(part 1 of 2)
# Autodesk Inventor assembly: gasienica_zlozenie
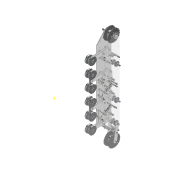
[picture p0: Inventor's stored thumbnail of the model, 180x180]
Saved by Autodesk Inventor 2020.3 (Build 243373000, 373)
## iProperties
Created: 2021-10-24
Part Number: gasienica_zlozenie
Document SubType Name: Assembly
Designer: Patryk Szydlik
Project: Projekt gąsienicowego układu jezdnego robota mobilnego "Ariadna"
Description: Projekt gąsienicowego układu jezdnego robota mobilnego "Ariadna"
Author: Patryk Szydlik
Title: Projekt gąsienicowego układu jezdnego robota mobilnego "Ariadna"
Subject: Projekt gąsienicowego układu jezdnego robota mobilnego "Ariadna"
## Documents named in this file (46)
- C:\Users\patry\Desktop\Semestr 7\Inzynierka\Projekt inventor\Ariadna_inzynierka\Workspaces\Obszar roboczy\Obszar roboczy\Naped\Zawieszenie_v3\gasienica_zlozenie.iam
- C:\Users\patry\Desktop\Semestr 7\Inzynierka\Projekt inventor\Ariadna_inzynierka\Workspaces\Obszar roboczy\Obszar roboczy\Naped\Kola\kolo_przednie.iam
- C:\Users\patry\Desktop\Semestr 7\Inzynierka\Projekt inventor\Ariadna_inzynierka\Workspaces\Obszar roboczy\Obszar roboczy\Naped\Sruby\M5_nut_5mm.ipt
- C:\Users\patry\Desktop\Semestr 7\Inzynierka\Projekt inventor\Ariadna_inzynierka\Workspaces\Obszar roboczy\Obszar roboczy\Naped\Zawieszenie_v3\tuleja_TUF106040.ipt
- C:\Users\patry\Desktop\Semestr 7\Inzynierka\Projekt inventor\Ariadna_inzynierka\Workspaces\Obszar roboczy\Obszar roboczy\Naped\Sruby\M6_nut_5mm.ipt
- C:\Users\patry\Desktop\Semestr 7\Inzynierka\Projekt inventor\Ariadna_inzynierka\Workspaces\Obszar roboczy\Obszar roboczy\Naped\Amortyzator\Korpus.ipt
- C:\Users\patry\Desktop\Semestr 7\Inzynierka\Projekt inventor\Ariadna_inzynierka\Workspaces\Obszar roboczy\Obszar roboczy\Naped\Amortyzator\Tlok.ipt
- C:\Users\patry\Desktop\Semestr 7\Inzynierka\Projekt inventor\Ariadna_inzynierka\Workspaces\Obszar roboczy\Obszar roboczy\Naped\Amortyzator\Nakretka.ipt
- C:\Users\patry\Desktop\Semestr 7\Inzynierka\Projekt inventor\Ariadna_inzynierka\Workspaces\Obszar roboczy\Obszar roboczy\Naped\Sruby\M8_nut_6.5mm_MIR1.ipt
- C:\Users\patry\Desktop\Semestr 7\Inzynierka\Projekt inventor\Ariadna_inzynierka\Workspaces\Obszar roboczy\Obszar roboczy\Naped\Sruby\M8x80_threaded_MIR1.ipt
- C:\Users\patry\Desktop\Semestr 7\Inzynierka\Projekt inventor\Ariadna_inzynierka\Workspaces\Obszar roboczy\Obszar roboczy\Naped\Sruby\M8_pad_MIR1.ipt
- C:\Users\patry\Desktop\Semestr 7\Inzynierka\Projekt inventor\Ariadna_inzynierka\Workspaces\Obszar roboczy\Obszar roboczy\Naped\Lozyska\608ZZ-8mm\bearings-608zz-80018-1.snapshot.1\608zz_MIR1.ipt
- C:\Users\patry\Desktop\Semestr 7\Inzynierka\Projekt inventor\Ariadna_inzynierka\Workspaces\Obszar roboczy\Obszar roboczy\Naped\Kola\kolo_napedowe.iam
- C:\Users\patry\Desktop\Semestr 7\Inzynierka\Projekt inventor\Ariadna_inzynierka\Workspaces\Obszar roboczy\Obszar roboczy\Naped\Sruby\M5_70_shaft.ipt
- C:\Users\patry\Desktop\Semestr 7\Inzynierka\Projekt inventor\Ariadna_inzynierka\Workspaces\Obszar roboczy\Obszar roboczy\Naped\Sruby\M3_16_shaft.ipt
- C:\Users\patry\Desktop\Semestr 7\Inzynierka\Projekt inventor\Ariadna_inzynierka\Workspaces\Obszar roboczy\Obszar roboczy\Naped\Sruby\M3_nut_2,5mm.ipt
- C:\Users\patry\Desktop\Semestr 7\Inzynierka\Projekt inventor\Ariadna_inzynierka\Workspaces\Obszar roboczy\Obszar roboczy\Naped\Zawieszenie_v3\wspornik_amortyzatora.ipt
- C:\Users\patry\Desktop\Semestr 7\Inzynierka\Projekt inventor\Ariadna_inzynierka\Workspaces\Obszar roboczy\Obszar roboczy\Naped\Sruby\M6_70_shaft.ipt
- C:\Users\patry\Desktop\Semestr 7\Inzynierka\Projekt inventor\Ariadna_inzynierka\Workspaces\Obszar roboczy\Obszar roboczy\Naped\Sruby\tuleja_M5_M9_20.ipt
- C:\Users\patry\Desktop\Semestr 7\Inzynierka\Projekt inventor\Ariadna_inzynierka\Workspaces\Obszar roboczy\Obszar roboczy\Naped\Sruby\tuleja_M5_M9_25.ipt
- C:\Users\patry\Desktop\Semestr 7\Inzynierka\Projekt inventor\Ariadna_inzynierka\Workspaces\Obszar roboczy\Obszar roboczy\Naped\Kola\holder_wheel_pair.iam
- C:\Users\patry\Desktop\Semestr 7\Inzynierka\Projekt inventor\Ariadna_inzynierka\Workspaces\Obszar roboczy\Obszar roboczy\Naped\Zawieszenie_v3\ramie_napinacza.ipt
- C:\Users\patry\Desktop\Semestr 7\Inzynierka\Projekt inventor\Ariadna_inzynierka\Workspaces\Obszar roboczy\Obszar roboczy\Naped\Sruby\M5_60_shaft.ipt
- C:\Users\patry\Desktop\Semestr 7\Inzynierka\Projekt inventor\Ariadna_inzynierka\Workspaces\Obszar roboczy\Obszar roboczy\Naped\Sruby\tuleja_M5_M9_13.ipt
- C:\Users\patry\Desktop\Semestr 7\Inzynierka\Projekt inventor\Ariadna_inzynierka\Workspaces\Obszar roboczy\Obszar roboczy\Naped\Sruby\tuleja_M5_M9_18.ipt
- C:\Users\patry\Desktop\Semestr 7\Inzynierka\Projekt inventor\Ariadna_inzynierka\Workspaces\Obszar roboczy\Obszar roboczy\Naped\Sruby\tuleja_M6_M10_8.ipt
- C:\Users\patry\Desktop\Semestr 7\Inzynierka\Projekt inventor\Ariadna_inzynierka\Workspaces\Obszar roboczy\Obszar roboczy\Naped\Zawieszenie_v3\plyta_boczna.ipt
- C:\Users\patry\Desktop\Semestr 7\Inzynierka\Projekt inventor\Ariadna_inzynierka\Workspaces\Obszar roboczy\Obszar roboczy\Naped\Zawieszenie_v3\ramie_1_wahacza.ipt
- C:\Users\patry\Desktop\Semestr 7\Inzynierka\Projekt inventor\Ariadna_inzynierka\Workspaces\Obszar roboczy\Obszar roboczy\Naped\Zawieszenie_v3\ramie_2_wahacza.ipt
- C:\Users\patry\Desktop\Semestr 7\Inzynierka\Projekt inventor\Ariadna_inzynierka\Workspaces\Obszar roboczy\Obszar roboczy\Naped\Sruby\M6_40_shaft.ipt
- C:\Users\patry\Desktop\Semestr 7\Inzynierka\Projekt inventor\Ariadna_inzynierka\Workspaces\Obszar roboczy\Obszar roboczy\Naped\Sruby\tuleja_M6_M10_7.ipt
- C:\Users\patry\Desktop\Semestr 7\Inzynierka\Projekt inventor\Ariadna_inzynierka\Workspaces\Obszar roboczy\Obszar roboczy\Naped\Sruby\M6_1,25_pad.ipt
- C:\Users\patry\Desktop\Semestr 7\Inzynierka\Projekt inventor\Ariadna_inzynierka\Workspaces\Obszar roboczy\Obszar roboczy\Naped\Sruby\M5_40_shaft.ipt
- M5_shaft.ipt
- C:\Users\patry\Desktop\Semestr 7\Inzynierka\Projekt inventor\Ariadna_inzynierka\Workspaces\Obszar roboczy\Obszar roboczy\Naped\Sruby\tuleja_M5_M9_4,5.ipt
- C:\Users\patry\Desktop\Semestr 7\Inzynierka\Projekt inventor\Ariadna_inzynierka\Workspaces\Obszar roboczy\Obszar roboczy\Naped\Zawieszenie_v3\glowny_wahacz_zewn.ipt
- C:\Users\patry\Desktop\Semestr 7\Inzynierka\Projekt inventor\Ariadna_inzynierka\Workspaces\Obszar roboczy\Obszar roboczy\Naped\Zawieszenie_v3\independent_wheel_pair.iam
- C:\Users\patry\Desktop\Semestr 7\Inzynierka\Projekt inventor\Ariadna_inzynierka\Workspaces\Obszar roboczy\Obszar roboczy\Naped\Sruby\tuleja_M6_M10_6.ipt
- C:\Users\patry\Desktop\Semestr 7\Inzynierka\Projekt inventor\Ariadna_inzynierka\Workspaces\Obszar roboczy\Obszar roboczy\Naped\Sruby\tuleja_M5_M9_17.5.ipt
- C:\Users\patry\Desktop\Semestr 7\Inzynierka\Projekt inventor\Ariadna_inzynierka\Workspaces\Obszar roboczy\Obszar roboczy\Naped\Zawieszenie_v3\komplet_kol_V4.iam
- C:\Users\patry\Desktop\Semestr 7\Inzynierka\Projekt inventor\Ariadna_inzynierka\Workspaces\Obszar roboczy\Obszar roboczy\Naped\Sruby\M6_25_shaft.ipt
- C:\Users\patry\Desktop\Semestr 7\Inzynierka\Projekt inventor\Ariadna_inzynierka\Workspaces\Obszar roboczy\Obszar roboczy\Naped\Kola\single_wheel_dummie.iam
- C:\Users\patry\Desktop\Semestr 7\Inzynierka\Projekt inventor\Ariadna_inzynierka\Workspaces\Obszar roboczy\Obszar roboczy\Naped\Sruby\tuleja_M5_M10_15.ipt
- C:\Users\patry\Desktop\Semestr 7\Inzynierka\Projekt inventor\Ariadna_inzynierka\Workspaces\Obszar roboczy\Obszar roboczy\Naped\Sruby\tuleja_M6_M10_7,5.ipt
- C:\Users\patry\Desktop\Semestr 7\Inzynierka\Projekt inventor\Ariadna_inzynierka\Workspaces\Obszar roboczy\Obszar roboczy\Naped\Zawieszenie_v3\ramie_2_wahacza_tylnego.ipt
- C:\Users\patry\Desktop\Semestr 7\Inzynierka\Projekt inventor\Ariadna_inzynierka\Workspaces\Obszar roboczy\Obszar roboczy\Naped\Sruby\M6x25_plaski_leb.ipt
## Components (343 placed, 44 different names)
1. M8_nut_6.5mm_MIR1:1
2. M8x80_threaded_MIR1:1
3. M8_nut_6.5mm_MIR1:2
4. M8_nut_6.5mm_MIR1:3
5. M8_pad_MIR1:1
6. M8_pad_MIR1:2
7. M8_pad_MIR1:3
8. M8_pad_MIR1:4
9. 608zz_MIR1:1
10. 608zz_MIR1:2 — Zestawiające:1077, Równoległe:74
11. kolo_napedowe:1 [sub-assembly]
12. kolo_przednie:1 [sub-assembly]
13. ramie_napinacza:1 — Zestawiające:1807
14. Korpus:6 — Walcowe:6
15. Tlok:6 — Walcowe:6
16. Nakretka:6
17. M5_nut_5mm:34
18. M5_70_shaft:6 — Zestawiające:1080
19. M5_nut_5mm:35
20. M3_16_shaft:6
21. M3_nut_2,5mm:11
22. M3_nut_2,5mm:12
23. wspornik_amortyzatora:11 — Zestawiające:1086, Zestawiające:1087
24. wspornik_amortyzatora:12
25. M5_nut_5mm:36
26. M5_nut_5mm:37
27. M5_nut_5mm:38
28. M5_nut_5mm:39
29. tuleja_M5_M9_20:6
30. tuleja_M5_M9_25:6
31. ramie_napinacza:2 — Zestawiające:1804
32. M5_60_shaft:1 — Zestawiające:1086
33. M5_60_shaft:2 — Zestawiające:1087, Zestawiające:1796, Zestawiające:1797
34. tuleja_TUF106040:41 — Zestawiające:1085
35. tuleja_TUF106040:42
36. M6_70_shaft:11 — Zestawiające:1079, Zestawiające:1802, Zestawiające:1803, Zestawiające:1806
37. M6_nut_5mm:49
38. M6_nut_5mm:50
39. tuleja_M5_M9_13:1 — Zestawiające:1796
40. tuleja_M5_M9_18:1 — Zestawiające:1797
41. M6_70_shaft:12
42. M6_nut_5mm:51
43. M6_nut_5mm:52
44. tuleja_M6_M10_8:1
45. tuleja_M6_M10_8:2
46. holder_wheel_pair:4 [sub-assembly] — Zestawiające:1082, Zestawiające:1083
47. holder_wheel_pair:5 [sub-assembly] — Zestawiające:1081, Zestawiające:1084
48. plyta_boczna:1 — Zestawiające:1075, Zestawiające:1076, Zestawiające:1077, Zestawiające:1078, Równoległe:74, Kątowe:22, Zestawiające:1079, Zestawiające:1080, Zestawiające:1081, Zestawiające:1082, Zestawiające:1083, Zestawiające:1084, Zestawiające:1085, Zestawiające:1632, Zestawiające:1633, Kątowe:49, Zestawiające:1950, Zestawiające:1951, Zestawiające:1952, Zestawiające:1953
49. plyta_boczna:2 — Zestawiające:1075, Zestawiające:1076, Zestawiające:1078, Zestawiające:1636, Zestawiające:1637, Zestawiające:1638, Zestawiające:1639, Zestawiające:1640, Zestawiające:1641, Zestawiające:1777, Zestawiające:1778, Zestawiające:1779, Zestawiające:1780
50. ramie_1_wahacza:3
51. ramie_2_wahacza:3
52. tuleja_TUF106040:51
53. tuleja_TUF106040:52
54. tuleja_TUF106040:53
55. tuleja_TUF106040:54
56. tuleja_TUF106040:55
57. tuleja_TUF106040:56
58. ramie_2_wahacza:4
59. tuleja_TUF106040:57
60. tuleja_TUF106040:58
61. M6_nut_5mm:65
62. Korpus:8
63. Tlok:8
64. Nakretka:8
65. M5_nut_5mm:48
66. M5_70_shaft:8
67. ramie_1_wahacza:4 — Kątowe:40
68. M5_nut_5mm:49
69. M3_16_shaft:8
70. M3_nut_2,5mm:15
71. M3_nut_2,5mm:16
72. wspornik_amortyzatora:15
73. wspornik_amortyzatora:16
74. M6_40_shaft:3
75. M6_40_shaft:4
76. M6_nut_5mm:66
77. M6_nut_5mm:67
78. M6_nut_5mm:68
79. tuleja_M6_M10_7:4
80. tuleja_M6_M10_7:5
81. M6_1,25_pad:9
82. M6_1,25_pad:10
83. M6_1,25_pad:11
84. M6_1,25_pad:12
85. M6_1,25_pad:13
86. M6_1,25_pad:14
87. M6_1,25_pad:15
88. M6_1,25_pad:16
89. M6_70_shaft:15 — Zestawiające:1636
90. M6_70_shaft:16 — Zestawiające:1632
91. M6_nut_5mm:69
92. M6_nut_5mm:70
93. M6_nut_5mm:71
94. M6_nut_5mm:72
95. M5_shaft:3
96. M5_shaft:4
97. M5_nut_5mm:50
98. M5_nut_5mm:51
99. M5_nut_5mm:52
100. M5_nut_5mm:53
101. tuleja_M5_M9_4,5:5
102. tuleja_M5_M9_4,5:6
103. tuleja_M5_M9_4,5:7
104. tuleja_M5_M9_4,5:8
105. lacznik_zewn:3 — Kątowe:40, Zestawiające:1793, Zestawiające:1794, Zestawiające:1795
106. lacznik_zewn:4 — Zestawiające:1793
107. tuleja_M6_M10_6:5
108. M6_nut_5mm:73
109. M6_nut_5mm:74
110. M6_nut_5mm:75 — Zestawiające:1633
111. M6_nut_5mm:76
112. tuleja_M6_M10_6:6
113. tuleja_M6_M10_6:7
114. tuleja_M6_M10_6:8
115. M5_nut_5mm:54
116. M5_nut_5mm:55
117. tuleja_M5_M9_17.5:3 — Zestawiające:1637
118. tuleja_M5_M9_17.5:4
119. ramie_1_wahacza:7 — Kątowe:41
120. ramie_2_wahacza:7
121. tuleja_TUF106040:67
122. tuleja_TUF106040:68
123. tuleja_TUF106040:69
124. tuleja_TUF106040:70
125. tuleja_TUF106040:71
126. tuleja_TUF106040:72
127. ramie_2_wahacza:8
128. tuleja_TUF106040:73
129. tuleja_TUF106040:74
130. M6_nut_5mm:89
131. Korpus:10 — Walcowe:10
132. Tlok:10 — Walcowe:10
133. Nakretka:10
134. M5_nut_5mm:64
135. M5_70_shaft:10
136. ramie_1_wahacza:8
137. M5_nut_5mm:65 — Zestawiające:1638
138. M3_16_shaft:10
139. M3_nut_2,5mm:19
140. M3_nut_2,5mm:20
141. wspornik_amortyzatora:19
142. wspornik_amortyzatora:20
143. M6_40_shaft:7
144. M6_40_shaft:8
145. M6_nut_5mm:90
146. M6_nut_5mm:91
147. M6_nut_5mm:92
148. tuleja_M6_M10_7:10
149. tuleja_M6_M10_7:11
150. M6_1,25_pad:25
151. M6_1,25_pad:26
152. M6_1,25_pad:27
153. M6_1,25_pad:28
154. M6_1,25_pad:29
155. M6_1,25_pad:30
156. M6_1,25_pad:31
157. M6_1,25_pad:32
158. M6_70_shaft:19 — Zestawiające:1640
159. M6_70_shaft:20 — Zestawiające:1639
160. M6_nut_5mm:93
161. M6_nut_5mm:94
162. M6_nut_5mm:95
163. M6_nut_5mm:96
164. M5_shaft:7
165. M5_shaft:8
166. M5_nut_5mm:66
167. M5_nut_5mm:67
168. M5_nut_5mm:68
169. M5_nut_5mm:69
170. tuleja_M5_M9_4,5:13
171. tuleja_M5_M9_4,5:14
172. tuleja_M5_M9_4,5:15
173. tuleja_M5_M9_4,5:16
174. lacznik_zewn:7 — Zestawiające:1784
175. lacznik_zewn:8 — Kątowe:41, Zestawiające:1781, Zestawiające:1782, Zestawiające:1789
176. tuleja_M6_M10_6:13
177. M6_nut_5mm:97
178. M6_nut_5mm:98
179. M6_nut_5mm:99
180. M6_nut_5mm:100
181. tuleja_M6_M10_6:14
182. tuleja_M6_M10_6:15
183. tuleja_M6_M10_6:16
184. M5_nut_5mm:70
185. M5_nut_5mm:71
186. tuleja_M5_M9_17.5:7 — Zestawiające:1641
187. tuleja_M5_M9_17.5:8
188. ramie_1_wahacza:9 — Kątowe:47
189. ramie_2_wahacza:9
190. tuleja_TUF106040:75
191. tuleja_TUF106040:76
192. tuleja_TUF106040:77
193. tuleja_TUF106040:78
194. tuleja_TUF106040:79
195. tuleja_TUF106040:80
196. ramie_2_wahacza:10
197. tuleja_TUF106040:81
198. tuleja_TUF106040:82
199. M6_nut_5mm:101
200. Korpus:11 — Walcowe:11
201. Tlok:11 — Walcowe:11
202. Nakretka:11
203. M5_nut_5mm:72
204. M5_70_shaft:11
205. ramie_1_wahacza:10
206. M5_nut_5mm:73
207. M3_16_shaft:11
208. M3_nut_2,5mm:21
209. M3_nut_2,5mm:22
210. wspornik_amortyzatora:21
211. wspornik_amortyzatora:22
212. M6_40_shaft:9
213. M6_40_shaft:10
214. M6_nut_5mm:102
215. M6_nut_5mm:103
216. M6_nut_5mm:104
217. tuleja_M6_M10_7:13
218. tuleja_M6_M10_7:14
219. M6_1,25_pad:33
220. M6_1,25_pad:34
221. M6_1,25_pad:35
222. M6_1,25_pad:36
223. M6_1,25_pad:37
224. M6_1,25_pad:38
225. M6_1,25_pad:39
226. M6_1,25_pad:40
227. M6_70_shaft:21 — Zestawiające:1779
228. M6_70_shaft:22 — Zestawiające:1778
229. M6_nut_5mm:105
230. M6_nut_5mm:106
231. M6_nut_5mm:107 — Zestawiające:1777
232. M6_nut_5mm:108
233. M5_shaft:9
234. M5_shaft:10
235. M5_nut_5mm:74
236. M5_nut_5mm:75
237. M5_nut_5mm:76
238. M5_nut_5mm:77
239. tuleja_M5_M9_4,5:17
240. tuleja_M5_M9_4,5:18
241. tuleja_M5_M9_4,5:19
242. tuleja_M5_M9_4,5:20
243. lacznik_zewn:9
244. lacznik_zewn:10 — Kątowe:47
245. independent_wheel_pair:5 [sub-assembly]
246. tuleja_M6_M10_7:15
247. tuleja_M6_M10_6:17
248. M6_nut_5mm:109
249. M6_nut_5mm:110
250. M6_nut_5mm:111
251. M6_nut_5mm:112
252. tuleja_M6_M10_6:18
253. tuleja_M6_M10_6:19
254. tuleja_M6_M10_6:20
255. M5_nut_5mm:78
256. M5_nut_5mm:79
257. tuleja_M5_M9_17.5:9
258. tuleja_M5_M9_17.5:10 — Zestawiające:1780
259. komplet_kol_V4:1 [sub-assembly] — Zestawiające:1781, Zestawiające:1782, Zestawiające:1784, Zestawiające:1788, Kątowe:48
260. M6_nut_5mm:115 — Zestawiające:1789
261. M6_25_shaft:2 — Zestawiające:1788
262. M6_nut_5mm:116
263. komplet_kol_V4:2 [sub-assembly] — Zestawiające:1795, Kątowe:48, Kątowe:49, Styczny:1
264. M6_nut_5mm:117
265. M6_25_shaft:3 — Zestawiające:1794
266. M6_nut_5mm:118
267. single_wheel_dummie:1 [sub-assembly] — Zestawiające:1799
268. single_wheel_dummie:2 [sub-assembly] — Zestawiające:1800, Zestawiające:1801, Zestawiające:1802, Zestawiające:1805
269. tuleja_M5_M10_15:1 — Zestawiające:1799, Zestawiające:1800, Zestawiające:1801
270. tuleja_M6_M10_7,5:1 — Zestawiające:1803, Zestawiające:1804, Zestawiające:1805
271. tuleja_M6_M10_7,5:2 — Zestawiające:1806, Zestawiające:1807
272. ramie_1_wahacza:11
273. tuleja_TUF106040:83
274. tuleja_TUF106040:84
275. tuleja_TUF106040:85
276. tuleja_TUF106040:86
277. tuleja_TUF106040:87
278. tuleja_TUF106040:88
279. tuleja_TUF106040:89
280. tuleja_TUF106040:90
281. M6_nut_5mm:119
282. Korpus:12 — Walcowe:12
283. Tlok:12 — Walcowe:12
284. Nakretka:12
285. M5_nut_5mm:80
286. M5_70_shaft:12
287. ramie_1_wahacza:12
288. M5_nut_5mm:81
289. M3_16_shaft:12
290. M3_nut_2,5mm:23
291. M3_nut_2,5mm:24
292. wspornik_amortyzatora:23
293. wspornik_amortyzatora:24
294. M6_40_shaft:11
295. M6_40_shaft:12
296. M6_nut_5mm:120
297. M6_nut_5mm:121
298. M6_nut_5mm:122
299. tuleja_M6_M10_7:16
300. tuleja_M6_M10_7:17
301. M6_1,25_pad:41
302. M6_1,25_pad:42
303. M6_1,25_pad:43
304. M6_1,25_pad:44
305. M6_1,25_pad:45
306. M6_1,25_pad:46
307. M6_1,25_pad:47
308. M6_1,25_pad:48
309. M6_70_shaft:23 — Zestawiające:1950
310. M6_nut_5mm:123 — Zestawiające:1951
311. M6_nut_5mm:124
312. M6_nut_5mm:125
313. M6_nut_5mm:126
314. M5_shaft:11
315. M5_shaft:12
316. M5_nut_5mm:82
317. M5_nut_5mm:83
318. M5_nut_5mm:84
319. M5_nut_5mm:85
320. tuleja_M5_M9_4,5:21
321. tuleja_M5_M9_4,5:22
322. tuleja_M5_M9_4,5:23
323. tuleja_M5_M9_4,5:24
324. lacznik_zewn:11
325. lacznik_zewn:12
326. independent_wheel_pair:6 [sub-assembly] — Styczny:1
327. tuleja_M6_M10_7:18
328. tuleja_M6_M10_6:21
329. M6_nut_5mm:127
330. M6_nut_5mm:128
331. M6_nut_5mm:129
332. M6_nut_5mm:130
333. tuleja_M6_M10_6:22 — Zestawiające:1952
334. tuleja_M6_M10_6:23
335. tuleja_M6_M10_6:24
336. M5_nut_5mm:86
337. M5_nut_5mm:87
338. tuleja_M5_M9_17.5:11
339. tuleja_M5_M9_17.5:12 — Zestawiające:1953
340. ramie_2_wahacza_tylnego:1
341. ramie_2_wahacza_tylnego:2
342. M6x25_plaski_leb:1
343. M6x25_plaski_leb:2
## Relationships (738: Mate 664, Flush 48, Angle 21, CylindricalJoint 4, Tangent 1)
- [Mate]: M8_nut_6.5mm_MIR1:1 ↔ M8x80_threaded_MIR1:1
- [Mate]: M8x80_threaded_MIR1:1 ↔ M8_nut_6.5mm_MIR1:2
- [Mate]: M8x80_threaded_MIR1:1 ↔ M8_nut_6.5mm_MIR1:3
- [Mate]: M8_nut_6.5mm_MIR1:1 ↔ M8_pad_MIR1:1
- [Mate] (7 mm): M8x80_threaded_MIR1:1 ↔ M8_pad_MIR1:1
- [Mate]: M8x80_threaded_MIR1:1 ↔ M8_pad_MIR1:1
- [Mate]: M8_nut_6.5mm_MIR1:1 ↔ M8_pad_MIR1:2
- [Mate]: M8x80_threaded_MIR1:1 ↔ M8_pad_MIR1:2
- [Mate] (7 mm): M8_nut_6.5mm_MIR1:2 ↔ M8_pad_MIR1:3
- [Mate]: M8_nut_6.5mm_MIR1:3 ↔ M8_pad_MIR1:3
- [Mate]: M8x80_threaded_MIR1:1 ↔ M8_pad_MIR1:3
- [Mate]: M8_nut_6.5mm_MIR1:3 ↔ M8_pad_MIR1:4
- [Mate] (31 mm): M8_pad_MIR1:2 ↔ M8_pad_MIR1:4
- [Mate]: M8x80_threaded_MIR1:1 ↔ M8_pad_MIR1:4
- [Mate]: M8x80_threaded_MIR1:1 ↔ 608zz_MIR1:1
- [Mate]: M8_nut_6.5mm_MIR1:2 ↔ 608zz_MIR1:1
- [Mate]: M8x80_threaded_MIR1:1 ↔ 608zz_MIR1:2
- [Mate]: M8x80_threaded_MIR1:1 ↔ 608zz_MIR1:2
- [Mate]: M8x80_threaded_MIR1:1 ↔ kolo_napedowe:1
- [Mate]: M8_pad_MIR1:2 ↔ kolo_napedowe:1
- [Mate]: Korpus:6 ↔ Tlok:6
- [Angle] (0 deg): Korpus:6 ↔ Tlok:6
- [Mate]: Korpus:6 ↔ Nakretka:6
- [Mate] (5 mm): Korpus:6 ↔ Nakretka:6
- Walcowe:6 [CylindricalJoint]: Korpus:6 ↔ Tlok:6
- [Mate]: Korpus:6 ↔ M5_70_shaft:6
- [Flush] (-30 mm): Korpus:6 ↔ M5_70_shaft:6
- [Mate]: M5_nut_5mm:34 ↔ M5_70_shaft:6
- [Mate]: M5_70_shaft:6 ↔ M5_nut_5mm:35
- [Mate] (60 mm): M5_nut_5mm:34 ↔ M5_nut_5mm:35
- [Mate] (30 mm): Korpus:6 ↔ M5_nut_5mm:34
- [Mate]: wspornik_amortyzatora:11 ↔ wspornik_amortyzatora:12
- [Mate]: wspornik_amortyzatora:11 ↔ wspornik_amortyzatora:12
- [Mate] (5 mm): wspornik_amortyzatora:11 ↔ wspornik_amortyzatora:12
- [Mate]: M3_16_shaft:6 ↔ wspornik_amortyzatora:12
- [Flush] (-2.5 mm): M3_16_shaft:6 ↔ wspornik_amortyzatora:11
- [Mate]: M3_16_shaft:6 ↔ M3_nut_2,5mm:11
- [Mate]: M3_nut_2,5mm:11 ↔ wspornik_amortyzatora:11
- [Mate]: M3_16_shaft:6 ↔ M3_nut_2,5mm:12
- [Mate]: M3_nut_2,5mm:12 ↔ wspornik_amortyzatora:12
- [Mate]: Tlok:6 ↔ M3_16_shaft:6
- [Mate]: Tlok:6 ↔ wspornik_amortyzatora:12
- [Mate]: M5_70_shaft:6 ↔ tuleja_M5_M9_20:6
- [Mate]: Korpus:6 ↔ tuleja_M5_M9_20:6
- [Mate]: M5_70_shaft:6 ↔ tuleja_M5_M9_25:6
- [Mate]: Korpus:6 ↔ tuleja_M5_M9_25:6
- [Mate]: M6_70_shaft:11 ↔ M6_nut_5mm:49
- [Mate]: M6_70_shaft:11 ↔ M6_nut_5mm:50
- [Mate] (60 mm): M6_nut_5mm:49 ↔ M6_nut_5mm:50
- [Mate]: tuleja_TUF106040:41 ↔ M6_70_shaft:11
- [Mate]: ramie_napinacza:1 ↔ ramie_napinacza:2
- [Mate]: ramie_napinacza:1 ↔ ramie_napinacza:2
- [Mate] (42 mm): ramie_napinacza:1 ↔ ramie_napinacza:2
- [Mate]: ramie_napinacza:1 ↔ tuleja_TUF106040:41
- [Mate]: ramie_napinacza:1 ↔ tuleja_TUF106040:41
- [Mate]: ramie_napinacza:2 ↔ tuleja_TUF106040:42
- [Mate]: ramie_napinacza:2 ↔ tuleja_TUF106040:42
- [Mate] (5 mm): tuleja_TUF106040:41 ↔ M6_nut_5mm:49
- [Flush] (-11 mm): ramie_napinacza:2 ↔ M6_70_shaft:11
- [Mate] (5.5 mm): kolo_przednie:1 ↔ ramie_napinacza:1
- [Mate]: kolo_przednie:1 ↔ ramie_napinacza:1
- [Mate]: ramie_napinacza:1 ↔ M5_60_shaft:1
- [Flush] (6 mm): ramie_napinacza:1 ↔ M5_60_shaft:1
- [Mate]: ramie_napinacza:1 ↔ M5_60_shaft:2
- [Flush] (6 mm): ramie_napinacza:1 ↔ M5_60_shaft:2
- [Mate]: M5_nut_5mm:37 ↔ M5_60_shaft:1
- [Mate]: ramie_napinacza:1 ↔ M5_nut_5mm:37
- [Mate]: M5_nut_5mm:38 ↔ M5_60_shaft:1
- [Mate]: M5_nut_5mm:38 ↔ ramie_napinacza:2
- [Mate]: M5_nut_5mm:39 ↔ M5_60_shaft:2
- [Mate]: M5_nut_5mm:39 ↔ ramie_napinacza:2
- [Mate]: M5_nut_5mm:36 ↔ M5_60_shaft:2
- [Mate]: ramie_napinacza:1 ↔ M5_nut_5mm:36
- [Flush]: M5_nut_5mm:34 ↔ M6_nut_5mm:50
- [Mate]: wspornik_amortyzatora:12 ↔ tuleja_M5_M9_18:1
- [Mate]: ramie_napinacza:1 ↔ tuleja_M5_M9_13:1
- [Mate]: ramie_napinacza:1 ↔ M6_70_shaft:12
- [Flush] (-11 mm): ramie_napinacza:1 ↔ M6_70_shaft:12
- [Mate]: M6_70_shaft:12 ↔ M6_nut_5mm:51
- [Mate]: ramie_napinacza:1 ↔ M6_nut_5mm:51
- [Mate]: M6_70_shaft:12 ↔ M6_nut_5mm:52
- [Mate]: ramie_napinacza:2 ↔ M6_nut_5mm:52
- [Mate]: M6_70_shaft:12 ↔ tuleja_M6_M10_8:1
- [Mate]: ramie_napinacza:1 ↔ tuleja_M6_M10_8:1
- [Mate]: M6_70_shaft:12 ↔ tuleja_M6_M10_8:2
- [Mate]: ramie_napinacza:2 ↔ tuleja_M6_M10_8:2
- Zestawiające:1075 [Mate]: plyta_boczna:1 ↔ plyta_boczna:2
- Zestawiające:1076 [Mate]: plyta_boczna:1 ↔ plyta_boczna:2
- Zestawiające:1077 [Mate]: 608zz_MIR1:2 ↔ plyta_boczna:1
- Zestawiające:1078 [Mate] (50 mm): plyta_boczna:1 ↔ plyta_boczna:2
- Równoległe:74 [Flush] (-1 mm): 608zz_MIR1:2 ↔ plyta_boczna:1
- Kątowe:22 [Angle] (180 deg): plyta_boczna:1
- Zestawiające:1079 [Mate]: M6_70_shaft:11 ↔ plyta_boczna:1
- Zestawiające:1080 [Mate]: M5_70_shaft:6 ↔ plyta_boczna:1
- Zestawiające:1081 [Mate]: holder_wheel_pair:5 ↔ plyta_boczna:1
- Zestawiające:1082 [Mate]: holder_wheel_pair:4 ↔ plyta_boczna:1
- Zestawiające:1083 [Mate]: holder_wheel_pair:4 ↔ plyta_boczna:1
- Zestawiające:1084 [Mate]: holder_wheel_pair:5 ↔ plyta_boczna:1
- Zestawiające:1085 [Mate]: tuleja_TUF106040:41 ↔ plyta_boczna:1
- Zestawiające:1086 [Mate]: wspornik_amortyzatora:11 ↔ M5_60_shaft:1
- Zestawiające:1087 [Mate]: wspornik_amortyzatora:11 ↔ M5_60_shaft:2
- [Mate]: ramie_2_wahacza:3 ↔ tuleja_TUF106040:51
- [Mate]: ramie_2_wahacza:3 ↔ tuleja_TUF106040:51
- [Angle] (0 deg): ramie_2_wahacza:3 ↔ tuleja_TUF106040:51
- [Mate]: ramie_1_wahacza:3 ↔ tuleja_TUF106040:54
- [Mate]: ramie_1_wahacza:3 ↔ tuleja_TUF106040:54
- [Angle] (0 deg): ramie_1_wahacza:3 ↔ tuleja_TUF106040:54
- [Mate]: ramie_2_wahacza:4 ↔ tuleja_TUF106040:57
- [Mate]: ramie_2_wahacza:4 ↔ tuleja_TUF106040:57
- [Angle] (0 deg): ramie_2_wahacza:4 ↔ tuleja_TUF106040:57
- [Mate]: Korpus:8 ↔ Tlok:8
- [Angle] (0 deg): Korpus:8 ↔ Tlok:8
- [Mate]: Korpus:8 ↔ Nakretka:8
- [Mate] (5 mm): Korpus:8 ↔ Nakretka:8
- [Mate]: Korpus:8 ↔ M5_70_shaft:8
- [Flush] (-32.5 mm): Korpus:8 ↔ M5_70_shaft:8
- [Mate]: M5_nut_5mm:48 ↔ M5_70_shaft:8
- [Mate]: M5_70_shaft:8 ↔ M5_nut_5mm:49
- [Mate] (60 mm): M5_nut_5mm:48 ↔ M5_nut_5mm:49
- [Mate] (27.5 mm): Korpus:8 ↔ M5_nut_5mm:48
- [Mate]: tuleja_TUF106040:56 ↔ ramie_1_wahacza:4
- [Mate]: tuleja_TUF106040:55 ↔ ramie_1_wahacza:4
- [Mate]: tuleja_TUF106040:56 ↔ ramie_1_wahacza:4
- [Mate]: tuleja_TUF106040:51 ↔ tuleja_TUF106040:57
- [Mate]: wspornik_amortyzatora:15 ↔ wspornik_amortyzatora:16
- [Mate]: wspornik_amortyzatora:15 ↔ wspornik_amortyzatora:16
- [Mate] (5 mm): wspornik_amortyzatora:15 ↔ wspornik_amortyzatora:16
- [Mate]: M3_16_shaft:8 ↔ wspornik_amortyzatora:16
- [Flush] (-2.5 mm): M3_16_shaft:8 ↔ wspornik_amortyzatora:15
- [Mate]: M3_16_shaft:8 ↔ M3_nut_2,5mm:15
- [Mate]: M3_nut_2,5mm:15 ↔ wspornik_amortyzatora:15
- [Mate]: M3_16_shaft:8 ↔ M3_nut_2,5mm:16
- [Mate]: M3_nut_2,5mm:16 ↔ wspornik_amortyzatora:16
- [Mate]: Tlok:8 ↔ M3_16_shaft:8
- [Mate]: Tlok:8 ↔ wspornik_amortyzatora:16
- [Mate]: ramie_1_wahacza:3 ↔ wspornik_amortyzatora:15
- [Mate]: ramie_1_wahacza:3 ↔ wspornik_amortyzatora:15
- [Mate] (4.5 mm): ramie_1_wahacza:3 ↔ wspornik_amortyzatora:15
- [Mate]: tuleja_TUF106040:54 ↔ M6_40_shaft:3
- [Flush] (7 mm): ramie_1_wahacza:3 ↔ M6_40_shaft:3
- [Mate]: tuleja_TUF106040:57 ↔ M6_40_shaft:4
- [Flush] (7 mm): ramie_2_wahacza:4 ↔ M6_40_shaft:4
- [Mate]: M6_nut_5mm:65 ↔ M6_40_shaft:3
- [Mate]: ramie_1_wahacza:3 ↔ M6_nut_5mm:65
- [Mate]: M6_40_shaft:3 ↔ M6_nut_5mm:66
- [Mate]: ramie_1_wahacza:4 ↔ M6_nut_5mm:66
- [Mate]: M6_40_shaft:4 ↔ M6_nut_5mm:67
- [Mate]: ramie_2_wahacza:3 ↔ M6_nut_5mm:67
- [Mate]: M6_40_shaft:4 ↔ M6_nut_5mm:68
- [Mate]: ramie_2_wahacza:4 ↔ M6_nut_5mm:68
- [Mate]: M6_40_shaft:3 ↔ tuleja_M6_M10_7:4
- [Mate]: M6_40_shaft:4 ↔ tuleja_M6_M10_7:5
- [Mate]: M6_1,25_pad:9 ↔ M6_1,25_pad:10
- [Mate]: M6_1,25_pad:9 ↔ M6_1,25_pad:10
- [Mate]: M6_40_shaft:3 ↔ M6_1,25_pad:9
- [Mate]: M6_1,25_pad:11 ↔ M6_1,25_pad:12
- [Mate]: M6_1,25_pad:11 ↔ M6_1,25_pad:12
- [Mate]: M6_40_shaft:3 ↔ M6_1,25_pad:11
- [Mate]: tuleja_TUF106040:54 ↔ M6_1,25_pad:11
- [Mate]: M6_1,25_pad:13 ↔ M6_1,25_pad:14
- [Mate]: M6_1,25_pad:13 ↔ M6_1,25_pad:14
- [Mate]: M6_40_shaft:4 ↔ M6_1,25_pad:13
- [Mate]: M6_1,25_pad:15 ↔ M6_1,25_pad:16
- [Mate]: M6_1,25_pad:15 ↔ M6_1,25_pad:16
- [Mate]: M6_40_shaft:4 ↔ M6_1,25_pad:15
- [Mate]: tuleja_TUF106040:57 ↔ M6_1,25_pad:15
- [Mate]: M5_70_shaft:8 ↔ M6_70_shaft:15
- [Flush]: M5_70_shaft:8 ↔ M6_70_shaft:16
- [Mate]: M6_70_shaft:16 ↔ M6_nut_5mm:69
- [Mate]: M6_70_shaft:16 ↔ M6_nut_5mm:70
- [Mate] (60 mm): M6_nut_5mm:69 ↔ M6_nut_5mm:70
- [Flush]: M5_nut_5mm:48 ↔ M6_nut_5mm:70
- [Mate] (60 mm): M6_nut_5mm:71 ↔ M6_nut_5mm:72
- [Mate]: M6_nut_5mm:71 ↔ M6_nut_5mm:72
- [Mate]: M6_70_shaft:15 ↔ M6_nut_5mm:71
- [Flush]: M5_nut_5mm:48 ↔ M6_nut_5mm:72
- [Mate]: ramie_1_wahacza:3 ↔ M5_shaft:3
- [Flush] (7 mm): ramie_1_wahacza:3 ↔ M5_shaft:3
- [Mate]: ramie_1_wahacza:3 ↔ M5_shaft:4
- [Flush] (7 mm): ramie_1_wahacza:3 ↔ M5_shaft:4
- [Mate]: M5_shaft:4 ↔ M5_nut_5mm:50
- [Mate]: ramie_1_wahacza:3 ↔ M5_nut_5mm:50
- [Mate]: M5_shaft:3 ↔ M5_nut_5mm:51
- [Mate]: ramie_1_wahacza:3 ↔ M5_nut_5mm:51
- [Mate]: M5_shaft:3 ↔ M5_nut_5mm:52
- [Mate]: ramie_1_wahacza:4 ↔ M5_nut_5mm:52
- [Mate]: M5_shaft:4 ↔ M5_nut_5mm:53
- [Mate]: ramie_1_wahacza:4 ↔ M5_nut_5mm:53
- [Mate]: M5_shaft:3 ↔ tuleja_M5_M9_4,5:5
- [Mate]: ramie_1_wahacza:4 ↔ tuleja_M5_M9_4,5:5
- [Mate]: M5_shaft:3 ↔ tuleja_M5_M9_4,5:6
- [Mate]: ramie_1_wahacza:3 ↔ tuleja_M5_M9_4,5:6
- [Mate]: M5_shaft:4 ↔ tuleja_M5_M9_4,5:7
- [Mate]: ramie_1_wahacza:4 ↔ tuleja_M5_M9_4,5:7
- [Mate]: M5_shaft:4 ↔ tuleja_M5_M9_4,5:8
- [Mate]: ramie_1_wahacza:3 ↔ tuleja_M5_M9_4,5:8
- [Mate]: M6_40_shaft:4 ↔ lacznik_zewn:3
- [Mate]: tuleja_M6_M10_7:5 ↔ lacznik_zewn:3
- [Mate]: M6_40_shaft:3 ↔ lacznik_zewn:3
- [Mate]: M6_40_shaft:4 ↔ lacznik_zewn:4
- [Mate]: M6_40_shaft:3 ↔ lacznik_zewn:4
- [Mate]: tuleja_TUF106040:56 ↔ M6_40_shaft:3
- [Mate]: M6_1,25_pad:12 ↔ lacznik_zewn:4
- [Mate]: M6_1,25_pad:16 ↔ lacznik_zewn:4
- [Mate]: tuleja_M6_M10_7:4 ↔ lacznik_zewn:3
- [Mate]: M6_1,25_pad:9 ↔ lacznik_zewn:3
- [Mate]: tuleja_TUF106040:56 ↔ M6_1,25_pad:10
- [Mate]: M6_1,25_pad:13 ↔ lacznik_zewn:3
- [Mate]: tuleja_TUF106040:51 ↔ M6_1,25_pad:14
- [Mate]: tuleja_TUF106040:55 ↔ ramie_1_wahacza:4
- [Mate]: tuleja_TUF106040:53 ↔ M6_70_shaft:16
- [Mate]: ramie_1_wahacza:3 ↔ tuleja_TUF106040:53
- [Mate]: ramie_1_wahacza:3 ↔ tuleja_TUF106040:53
- [Mate]: tuleja_TUF106040:52 ↔ M6_70_shaft:15
- [Mate]: ramie_2_wahacza:3 ↔ tuleja_TUF106040:52
- [Mate]: ramie_2_wahacza:3 ↔ tuleja_TUF106040:52
- [Mate]: tuleja_TUF106040:58 ↔ M6_70_shaft:15
- [Mate]: ramie_2_wahacza:4 ↔ tuleja_TUF106040:58
- [Mate]: ramie_2_wahacza:4 ↔ tuleja_TUF106040:58
- [Mate]: ramie_1_wahacza:4 ↔ M5_shaft:4
- [Mate]: M6_70_shaft:15 ↔ M6_nut_5mm:73
- [Mate] (5 mm): M6_nut_5mm:72 ↔ M6_nut_5mm:73
- [Mate]: M6_70_shaft:15 ↔ M6_nut_5mm:74
- [Mate] (5 mm): M6_nut_5mm:71 ↔ M6_nut_5mm:74
- [Mate]: M6_70_shaft:16 ↔ M6_nut_5mm:75
- [Mate] (5 mm): M6_nut_5mm:69 ↔ M6_nut_5mm:75
- [Mate]: M6_70_shaft:16 ↔ M6_nut_5mm:76
- [Mate] (5 mm): M6_nut_5mm:70 ↔ M6_nut_5mm:76
- [Mate]: M6_70_shaft:16 ↔ tuleja_M6_M10_6:5
- [Mate]: tuleja_M6_M10_6:5 ↔ M6_nut_5mm:75
- [Mate]: M6_70_shaft:15 ↔ tuleja_M6_M10_6:6
- [Mate]: tuleja_TUF106040:58 ↔ tuleja_M6_M10_6:6
- [Mate]: M6_70_shaft:15 ↔ tuleja_M6_M10_6:7
- [Mate]: tuleja_TUF106040:52 ↔ tuleja_M6_M10_6:7
- [Mate]: M6_70_shaft:16 ↔ tuleja_M6_M10_6:8
- [Mate]: tuleja_TUF106040:55 ↔ tuleja_M6_M10_6:8
- [Mate]: M5_70_shaft:8 ↔ M5_nut_5mm:54
- [Mate] (5 mm): M5_nut_5mm:48 ↔ M5_nut_5mm:54
- [Mate]: M5_70_shaft:8 ↔ M5_nut_5mm:55
- [Mate] (5 mm): M5_nut_5mm:49 ↔ M5_nut_5mm:55
- [Mate]: M5_70_shaft:8 ↔ tuleja_M5_M9_17.5:4
- [Mate]: M5_nut_5mm:55 ↔ tuleja_M5_M9_17.5:4
- [Mate]: M5_70_shaft:8 ↔ tuleja_M5_M9_17.5:3
- [Mate]: Korpus:8 ↔ tuleja_M5_M9_17.5:3
- [Mate]: ramie_2_wahacza:7 ↔ tuleja_TUF106040:67
- [Mate]: ramie_2_wahacza:7 ↔ tuleja_TUF106040:67
- [Angle] (0 deg): ramie_2_wahacza:7 ↔ tuleja_TUF106040:67
- [Mate]: ramie_1_wahacza:7 ↔ tuleja_TUF106040:70
- [Mate]: ramie_1_wahacza:7 ↔ tuleja_TUF106040:70
- [Angle] (0 deg): ramie_1_wahacza:7 ↔ tuleja_TUF106040:70
- [Mate]: ramie_2_wahacza:8 ↔ tuleja_TUF106040:73
- [Mate]: ramie_2_wahacza:8 ↔ tuleja_TUF106040:73
- [Angle] (0 deg): ramie_2_wahacza:8 ↔ tuleja_TUF106040:73
- [Mate]: Korpus:10 ↔ Tlok:10
- [Angle] (0 deg): Korpus:10 ↔ Tlok:10
- [Mate]: Korpus:10 ↔ Nakretka:10
- [Mate] (5 mm): Korpus:10 ↔ Nakretka:10
- Walcowe:10 [CylindricalJoint]: Korpus:10 ↔ Tlok:10
- [Mate]: Korpus:10 ↔ M5_70_shaft:10
- [Flush] (-32.5 mm): Korpus:10 ↔ M5_70_shaft:10
- [Mate]: M5_nut_5mm:64 ↔ M5_70_shaft:10
- [Mate]: M5_70_shaft:10 ↔ M5_nut_5mm:65
- [Mate] (60 mm): M5_nut_5mm:64 ↔ M5_nut_5mm:65
- [Mate] (27.5 mm): Korpus:10 ↔ M5_nut_5mm:64
- [Mate]: tuleja_TUF106040:72 ↔ ramie_1_wahacza:8
- [Mate]: tuleja_TUF106040:71 ↔ ramie_1_wahacza:8
- [Mate]: tuleja_TUF106040:72 ↔ ramie_1_wahacza:8
- [Mate]: tuleja_TUF106040:67 ↔ tuleja_TUF106040:73
- [Mate]: wspornik_amortyzatora:19 ↔ wspornik_amortyzatora:20
- [Mate]: wspornik_amortyzatora:19 ↔ wspornik_amortyzatora:20
- [Mate] (5 mm): wspornik_amortyzatora:19 ↔ wspornik_amortyzatora:20
- [Mate]: M3_16_shaft:10 ↔ wspornik_amortyzatora:20
- [Flush] (-2.5 mm): M3_16_shaft:10 ↔ wspornik_amortyzatora:19
- [Mate]: M3_16_shaft:10 ↔ M3_nut_2,5mm:19
- [Mate]: M3_nut_2,5mm:19 ↔ wspornik_amortyzatora:19
- [Mate]: M3_16_shaft:10 ↔ M3_nut_2,5mm:20
- [Mate]: M3_nut_2,5mm:20 ↔ wspornik_amortyzatora:20
- [Mate]: Tlok:10 ↔ M3_16_shaft:10
- [Mate]: Tlok:10 ↔ wspornik_amortyzatora:20
- [Mate]: ramie_1_wahacza:7 ↔ wspornik_amortyzatora:19
- [Mate]: ramie_1_wahacza:7 ↔ wspornik_amortyzatora:19
- [Mate] (4.5 mm): ramie_1_wahacza:7 ↔ wspornik_amortyzatora:19
- [Mate]: tuleja_TUF106040:70 ↔ M6_40_shaft:7
- [Flush] (7 mm): ramie_1_wahacza:7 ↔ M6_40_shaft:7
- [Mate]: tuleja_TUF106040:73 ↔ M6_40_shaft:8
- [Flush] (7 mm): ramie_2_wahacza:8 ↔ M6_40_shaft:8
- [Mate]: M6_nut_5mm:89 ↔ M6_40_shaft:7
- [Mate]: ramie_1_wahacza:7 ↔ M6_nut_5mm:89
- [Mate]: M6_40_shaft:7 ↔ M6_nut_5mm:90
- [Mate]: ramie_1_wahacza:8 ↔ M6_nut_5mm:90
- [Mate]: M6_40_shaft:8 ↔ M6_nut_5mm:91
- [Mate]: ramie_2_wahacza:7 ↔ M6_nut_5mm:91
- [Mate]: M6_40_shaft:8 ↔ M6_nut_5mm:92
- [Mate]: ramie_2_wahacza:8 ↔ M6_nut_5mm:92
- [Mate]: M6_40_shaft:7 ↔ tuleja_M6_M10_7:10
- [Mate]: M6_40_shaft:8 ↔ tuleja_M6_M10_7:11
- [Mate]: M6_1,25_pad:25 ↔ M6_1,25_pad:26
- [Mate]: M6_1,25_pad:25 ↔ M6_1,25_pad:26
- [Mate]: M6_40_shaft:7 ↔ M6_1,25_pad:25
- [Mate]: M6_1,25_pad:27 ↔ M6_1,25_pad:28
- [Mate]: M6_1,25_pad:27 ↔ M6_1,25_pad:28
- [Mate]: M6_40_shaft:7 ↔ M6_1,25_pad:27
- [Mate]: tuleja_TUF106040:70 ↔ M6_1,25_pad:27
- [Mate]: M6_1,25_pad:29 ↔ M6_1,25_pad:30
- [Mate]: M6_1,25_pad:29 ↔ M6_1,25_pad:30
- [Mate]: M6_40_shaft:8 ↔ M6_1,25_pad:29
- [Mate]: M6_1,25_pad:31 ↔ M6_1,25_pad:32
- [Mate]: M6_1,25_pad:31 ↔ M6_1,25_pad:32
- [Mate]: M6_40_shaft:8 ↔ M6_1,25_pad:31
- [Mate]: tuleja_TUF106040:73 ↔ M6_1,25_pad:31
- [Mate]: M5_70_shaft:10 ↔ M6_70_shaft:19
- [Flush]: M5_70_shaft:10 ↔ M6_70_shaft:20
- [Mate]: M6_70_shaft:20 ↔ M6_nut_5mm:93
- [Mate]: M6_70_shaft:20 ↔ M6_nut_5mm:94
- [Mate] (60 mm): M6_nut_5mm:93 ↔ M6_nut_5mm:94
- [Flush]: M5_nut_5mm:64 ↔ M6_nut_5mm:94
- [Mate] (60 mm): M6_nut_5mm:95 ↔ M6_nut_5mm:96
- [Mate]: M6_nut_5mm:95 ↔ M6_nut_5mm:96
- [Mate]: M6_70_shaft:19 ↔ M6_nut_5mm:95
- [Flush]: M5_nut_5mm:64 ↔ M6_nut_5mm:96
- [Mate]: ramie_1_wahacza:7 ↔ M5_shaft:7
- [Flush] (7 mm): ramie_1_wahacza:7 ↔ M5_shaft:7
- [Mate]: ramie_1_wahacza:7 ↔ M5_shaft:8
- [Flush] (7 mm): ramie_1_wahacza:7 ↔ M5_shaft:8
- [Mate]: M5_shaft:8 ↔ M5_nut_5mm:66
- [Mate]: ramie_1_wahacza:7 ↔ M5_nut_5mm:66
- [Mate]: M5_shaft:7 ↔ M5_nut_5mm:67
- [Mate]: ramie_1_wahacza:7 ↔ M5_nut_5mm:67
- [Mate]: M5_shaft:7 ↔ M5_nut_5mm:68
- [Mate]: ramie_1_wahacza:8 ↔ M5_nut_5mm:68
- [Mate]: M5_shaft:8 ↔ M5_nut_5mm:69
- [Mate]: ramie_1_wahacza:8 ↔ M5_nut_5mm:69
- [Mate]: M5_shaft:7 ↔ tuleja_M5_M9_4,5:13
- [Mate]: ramie_1_wahacza:8 ↔ tuleja_M5_M9_4,5:13
- [Mate]: M5_shaft:7 ↔ tuleja_M5_M9_4,5:14
- [Mate]: ramie_1_wahacza:7 ↔ tuleja_M5_M9_4,5:14
- [Mate]: M5_shaft:8 ↔ tuleja_M5_M9_4,5:15
- [Mate]: ramie_1_wahacza:8 ↔ tuleja_M5_M9_4,5:15
- [Mate]: M5_shaft:8 ↔ tuleja_M5_M9_4,5:16
- [Mate]: ramie_1_wahacza:7 ↔ tuleja_M5_M9_4,5:16
- [Mate]: M6_40_shaft:8 ↔ lacznik_zewn:7
- [Mate]: tuleja_M6_M10_7:11 ↔ lacznik_zewn:7
- [Mate]: M6_40_shaft:7 ↔ lacznik_zewn:7
- [Mate]: M6_40_shaft:8 ↔ lacznik_zewn:8
- [Mate]: M6_40_shaft:7 ↔ lacznik_zewn:8
- [Mate]: tuleja_TUF106040:72 ↔ M6_40_shaft:7
- [Mate]: M6_1,25_pad:28 ↔ lacznik_zewn:8
- [Mate]: M6_1,25_pad:32 ↔ lacznik_zewn:8
- [Mate]: tuleja_M6_M10_7:10 ↔ lacznik_zewn:7
- [Mate]: M6_1,25_pad:25 ↔ lacznik_zewn:7
- [Mate]: tuleja_TUF106040:72 ↔ M6_1,25_pad:26
- [Mate]: M6_1,25_pad:29 ↔ lacznik_zewn:7
- [Mate]: tuleja_TUF106040:67 ↔ M6_1,25_pad:30
- [Mate]: tuleja_TUF106040:71 ↔ ramie_1_wahacza:8
- [Mate]: tuleja_TUF106040:69 ↔ M6_70_shaft:20
- [Mate]: ramie_1_wahacza:7 ↔ tuleja_TUF106040:69
- [Mate]: ramie_1_wahacza:7 ↔ tuleja_TUF106040:69
- [Mate]: tuleja_TUF106040:68 ↔ M6_70_shaft:19
- [Mate]: ramie_2_wahacza:7 ↔ tuleja_TUF106040:68
- [Mate]: ramie_2_wahacza:7 ↔ tuleja_TUF106040:68
- [Mate]: tuleja_TUF106040:74 ↔ M6_70_shaft:19
- [Mate]: ramie_2_wahacza:8 ↔ tuleja_TUF106040:74
- [Mate]: ramie_2_wahacza:8 ↔ tuleja_TUF106040:74
- [Mate]: ramie_1_wahacza:8 ↔ M5_shaft:8
- [Mate]: M6_70_shaft:19 ↔ M6_nut_5mm:97
- [Mate] (5 mm): M6_nut_5mm:96 ↔ M6_nut_5mm:97
- [Mate]: M6_70_shaft:19 ↔ M6_nut_5mm:98
- [Mate] (5 mm): M6_nut_5mm:95 ↔ M6_nut_5mm:98
- [Mate]: M6_70_shaft:20 ↔ M6_nut_5mm:99
- [Mate] (5 mm): M6_nut_5mm:93 ↔ M6_nut_5mm:99
- [Mate]: M6_70_shaft:20 ↔ M6_nut_5mm:100
- [Mate] (5 mm): M6_nut_5mm:94 ↔ M6_nut_5mm:100
- [Mate]: M6_70_shaft:20 ↔ tuleja_M6_M10_6:13
- [Mate]: tuleja_M6_M10_6:13 ↔ M6_nut_5mm:99
- [Mate]: M6_70_shaft:19 ↔ tuleja_M6_M10_6:14
- [Mate]: tuleja_TUF106040:74 ↔ tuleja_M6_M10_6:14
- [Mate]: M6_70_shaft:19 ↔ tuleja_M6_M10_6:15
- [Mate]: tuleja_TUF106040:68 ↔ tuleja_M6_M10_6:15
- [Mate]: M6_70_shaft:20 ↔ tuleja_M6_M10_6:16
- [Mate]: tuleja_TUF106040:71 ↔ tuleja_M6_M10_6:16
- [Mate]: M5_70_shaft:10 ↔ M5_nut_5mm:70
- [Mate] (5 mm): M5_nut_5mm:64 ↔ M5_nut_5mm:70
- [Mate]: M5_70_shaft:10 ↔ M5_nut_5mm:71
- [Mate] (5 mm): M5_nut_5mm:65 ↔ M5_nut_5mm:71
- [Mate]: M5_70_shaft:10 ↔ tuleja_M5_M9_17.5:8
- [Mate]: M5_nut_5mm:71 ↔ tuleja_M5_M9_17.5:8
- [Mate]: M5_70_shaft:10 ↔ tuleja_M5_M9_17.5:7
- [Mate]: Korpus:10 ↔ tuleja_M5_M9_17.5:7
- Zestawiające:1632 [Mate]: plyta_boczna:1 ↔ M6_70_shaft:16
- Zestawiające:1633 [Mate]: plyta_boczna:1 ↔ M6_nut_5mm:75
- Zestawiające:1636 [Mate]: plyta_boczna:2 ↔ M6_70_shaft:15
- Zestawiające:1637 [Mate]: plyta_boczna:2 ↔ tuleja_M5_M9_17.5:3
- Kątowe:40 [Angle] (90 deg): ramie_1_wahacza:4 ↔ lacznik_zewn:3
- Zestawiające:1638 [Mate]: plyta_boczna:2 ↔ M5_nut_5mm:65
- Zestawiające:1639 [Mate]: plyta_boczna:2 ↔ M6_70_shaft:20
- Zestawiające:1640 [Mate]: plyta_boczna:2 ↔ M6_70_shaft:19
- Zestawiające:1641 [Mate]: plyta_boczna:2 ↔ tuleja_M5_M9_17.5:7
- Kątowe:41 [Angle] (90 deg): ramie_1_wahacza:7 ↔ lacznik_zewn:8
- [Mate]: ramie_2_wahacza:9 ↔ tuleja_TUF106040:75
- [Mate]: ramie_2_wahacza:9 ↔ tuleja_TUF106040:75
- [Angle] (0 deg): ramie_2_wahacza:9 ↔ tuleja_TUF106040:75
- [Mate]: ramie_1_wahacza:9 ↔ tuleja_TUF106040:78
- [Mate]: ramie_1_wahacza:9 ↔ tuleja_TUF106040:78
- [Angle] (0 deg): ramie_1_wahacza:9 ↔ tuleja_TUF106040:78
- [Mate]: ramie_2_wahacza:10 ↔ tuleja_TUF106040:81
- [Mate]: ramie_2_wahacza:10 ↔ tuleja_TUF106040:81
- [Angle] (0 deg): ramie_2_wahacza:10 ↔ tuleja_TUF106040:81
- [Mate]: Korpus:11 ↔ Tlok:11
- [Angle] (0 deg): Korpus:11 ↔ Tlok:11
- [Mate]: Korpus:11 ↔ Nakretka:11
- [Mate] (5 mm): Korpus:11 ↔ Nakretka:11
- Walcowe:11 [CylindricalJoint]: Korpus:11 ↔ Tlok:11
- [Mate]: Korpus:11 ↔ M5_70_shaft:11
- [Flush] (-32.5 mm): Korpus:11 ↔ M5_70_shaft:11
- [Mate]: M5_nut_5mm:72 ↔ M5_70_shaft:11
- [Mate]: M5_70_shaft:11 ↔ M5_nut_5mm:73
- [Mate] (60 mm): M5_nut_5mm:72 ↔ M5_nut_5mm:73
- [Mate] (27.5 mm): Korpus:11 ↔ M5_nut_5mm:72
- [Mate]: tuleja_TUF106040:80 ↔ ramie_1_wahacza:10
- [Mate]: tuleja_TUF106040:79 ↔ ramie_1_wahacza:10
- [Mate]: tuleja_TUF106040:80 ↔ ramie_1_wahacza:10
- [Mate]: tuleja_TUF106040:75 ↔ tuleja_TUF106040:81
- [Mate]: wspornik_amortyzatora:21 ↔ wspornik_amortyzatora:22
- [Mate]: wspornik_amortyzatora:21 ↔ wspornik_amortyzatora:22
- [Mate] (5 mm): wspornik_amortyzatora:21 ↔ wspornik_amortyzatora:22
- [Mate]: M3_16_shaft:11 ↔ wspornik_amortyzatora:22
- [Flush] (-2.5 mm): M3_16_shaft:11 ↔ wspornik_amortyzatora:21
- [Mate]: M3_16_shaft:11 ↔ M3_nut_2,5mm:21
- [Mate]: M3_nut_2,5mm:21 ↔ wspornik_amortyzatora:21
- [Mate]: M3_16_shaft:11 ↔ M3_nut_2,5mm:22
- [Mate]: M3_nut_2,5mm:22 ↔ wspornik_amortyzatora:22
- [Mate]: Tlok:11 ↔ M3_16_shaft:11
- [Mate]: Tlok:11 ↔ wspornik_amortyzatora:22